# Autodesk Inventor assembly: 000-hand-grab-v1
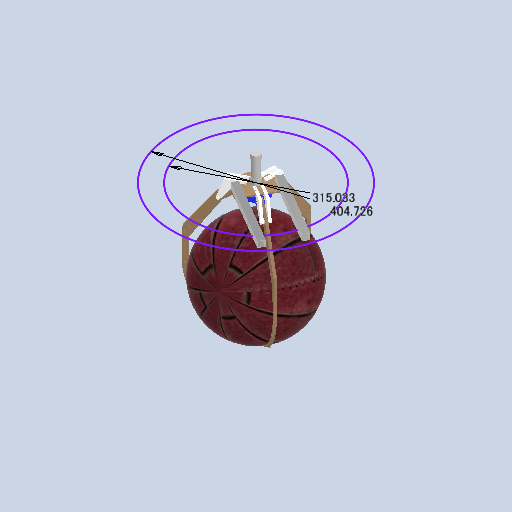
[picture p0: Inventor's stored thumbnail of the model, 512x512]
Saved by Autodesk Inventor 2025.1 (Build 291241000, 241)
## iProperties
Created: 2024-10-07
Part Number: 000-hand-grab-v1
Document SubType Name: Assembly
Designer: haruy
Author: haruy
## Documents named in this file (11)
- C:\Users\haruy\Documents\ロボコン\NHK2025\cad\nagahisa\hand\grab\000-hand-grab-v1.iam
- C:\Users\haruy\Documents\ロボコン\NHK2025\cad\nagahisa\hand\grab\hand-grab-v1-MDF-air-Base.ipt
- C:\Users\haruy\Documents\ロボコン\NHK2025\cad\nagahisa\hand\grab\hand-grab-v1-POM-link-F-1.ipt
- C:\Users\haruy\Documents\ロボコン\NHK2025\cad\nagahisa\hand\grab\hand-grab-v1-3DP-link-F-2.ipt
- C:\Users\haruy\Documents\ロボコン\NHK2025\cad\nagahisa\hand\grab\bearing-10-3.ipt
- C:\Users\haruy\Documents\ロボコン\NHK2025\cad\nagahisa\hand\grab\hand-grab-v1-POM-arm.ipt
- C:\Users\haruy\Documents\ロボコン\NHK2025\cad\nagahisa\hand\grab\C-SEFL683ZZ.ipt
- C:\Users\haruy\Documents\ロボコン\NHK2025\cad\nagahisa\hand\grab\E-NTBGT13-8.iam
- C:\Users\haruy\Documents\ロボコン\NHK2025\cad\basket-ball.ipt
- C:\Users\haruy\Documents\ロボコン\NHK2025\cad\000_parts\エアシリンダー\airclinder\CDJ2B16-15Z-B(0_1_0).iam
- C:\Users\haruy\Documents\ロボコン\NHK2025\cad\nagahisa\hand\grab\hand-grab-v1-ASP-arm-support.ipt
## Components (30 placed, 10 different names)
1. hand-grab-v1-MDF-air-Base:1 — 挿入:2, 挿入:3, 挿入:4, 挿入:5, 挿入:6, 挿入:7, 挿入:8, 挿入:9, 挿入:10, 挿入:11, 挿入:12, 挿入:13, 挿入:30, 挿入:32, 挿入:33, 挿入:34, 挿入:35
2. hand-grab-v1-POM-link-F-1:1 — 挿入:2, 挿入:3
3. hand-grab-v1-POM-link-F-1:2 — 挿入:4, 挿入:5
4. hand-grab-v1-POM-link-F-1:3 — 挿入:6, 挿入:7
5. hand-grab-v1-POM-link-F-1:4 — 挿入:8, 挿入:9
6. hand-grab-v1-POM-link-F-1:5 — 挿入:10, 挿入:11
7. hand-grab-v1-POM-link-F-1:6 — 挿入:12, 挿入:13, 角度:1, 挿入:29
8. hand-grab-v1-3DP-link-F-2:1 — 挿入:16, 挿入:18, 挿入:20, 角度:1, 挿入:31
9. bearing-10-3:1 — 挿入:15, 正接:3
10. bearing-10-3:2 — 挿入:15, 挿入:16
11. bearing-10-3:3
12. bearing-10-3:4 — 挿入:18
13. bearing-10-3:5 — 挿入:20
14. bearing-10-3:6
15. basket-ball:1 — 正接:4, 正接:5, 正接:6
16. CDJ2B16-15Z-B(0_1_0):1 [sub-assembly] — 挿入:30, 挿入:31
17. hand-grab-v1-ASP-arm-support:1 — 挿入:32, 挿入:34
18. hand-grab-v1-ASP-arm-support:2 — 挿入:33, 挿入:35
19. hand-grab-v1-POM-arm:1 — 挿入:26, 挿入:27, 挿入:28, 正接:3
20. E-NTBGT13-8:1 [sub-assembly] — 挿入:26, 正接:6
21. C-SEFL683ZZ:2 — 挿入:28
22. C-SEFL683ZZ:1 — 挿入:27, 挿入:29
23. hand-grab-v1-POM-arm:2
24. E-NTBGT13-8:2 [sub-assembly] — 正接:4
25. C-SEFL683ZZ:3
26. C-SEFL683ZZ:4
27. hand-grab-v1-POM-arm:3
28. E-NTBGT13-8:3 [sub-assembly] — 正接:5
29. C-SEFL683ZZ:5
30. C-SEFL683ZZ:6
## Component patterns: (3 elements, first: hand-grab-v1-POM-arm:1 + E-NTBGT13-8:1 + C-SEFL683ZZ:2 + C-SEFL683ZZ:1)
## Relationships (33: Insert 28, Tangent 4, Angle 1)
- 挿入:2 [Insert]: hand-grab-v1-MDF-air-Base:1 ↔ hand-grab-v1-POM-link-F-1:1
- 挿入:3 [Insert]: hand-grab-v1-MDF-air-Base:1 ↔ hand-grab-v1-POM-link-F-1:1
- 挿入:4 [Insert]: hand-grab-v1-MDF-air-Base:1 ↔ hand-grab-v1-POM-link-F-1:2
- 挿入:5 [Insert]: hand-grab-v1-MDF-air-Base:1 ↔ hand-grab-v1-POM-link-F-1:2
- 挿入:6 [Insert]: hand-grab-v1-MDF-air-Base:1 ↔ hand-grab-v1-POM-link-F-1:3
- 挿入:7 [Insert]: hand-grab-v1-MDF-air-Base:1 ↔ hand-grab-v1-POM-link-F-1:3
- 挿入:8 [Insert]: hand-grab-v1-MDF-air-Base:1 ↔ hand-grab-v1-POM-link-F-1:4
- 挿入:9 [Insert]: hand-grab-v1-MDF-air-Base:1 ↔ hand-grab-v1-POM-link-F-1:4
- 挿入:10 [Insert]: hand-grab-v1-MDF-air-Base:1 ↔ hand-grab-v1-POM-link-F-1:5
- 挿入:11 [Insert]: hand-grab-v1-MDF-air-Base:1 ↔ hand-grab-v1-POM-link-F-1:5
- 挿入:12 [Insert]: hand-grab-v1-MDF-air-Base:1 ↔ hand-grab-v1-POM-link-F-1:6
- 挿入:13 [Insert]: hand-grab-v1-MDF-air-Base:1 ↔ hand-grab-v1-POM-link-F-1:6
- 挿入:15 [Insert]: bearing-10-3:1 ↔ bearing-10-3:2
- 挿入:16 [Insert] (0.25 mm): hand-grab-v1-3DP-link-F-2:1 ↔ bearing-10-3:2
- [Insert]: bearing-10-3:3 ↔ bearing-10-3:4
- 挿入:18 [Insert] (0.25 mm): hand-grab-v1-3DP-link-F-2:1 ↔ bearing-10-3:4
- [Insert]: bearing-10-3:5 ↔ bearing-10-3:6
- 挿入:20 [Insert] (0.25 mm): hand-grab-v1-3DP-link-F-2:1 ↔ bearing-10-3:5
- 角度:1 [Angle] (0 deg): hand-grab-v1-POM-link-F-1:6 ↔ hand-grab-v1-3DP-link-F-2:1
- 挿入:26 [Insert]: hand-grab-v1-POM-arm:1 ↔ E-NTBGT13-8:1
- 挿入:27 [Insert]: hand-grab-v1-POM-arm:1 ↔ C-SEFL683ZZ:1
- 挿入:28 [Insert]: hand-grab-v1-POM-arm:1 ↔ C-SEFL683ZZ:2
- 挿入:29 [Insert] (0.2 mm): hand-grab-v1-POM-link-F-1:6 ↔ C-SEFL683ZZ:1
- 挿入:30 [Insert]: hand-grab-v1-MDF-air-Base:1 ↔ CDJ2B16-15Z-B(0_1_0):1
- 正接:3 [Tangent]: bearing-10-3:1 ↔ hand-grab-v1-POM-arm:1
- 正接:4 [Tangent]: basket-ball:1 ↔ E-NTBGT13-8:2
- 正接:5 [Tangent]: basket-ball:1 ↔ E-NTBGT13-8:3
- 正接:6 [Tangent]: basket-ball:1 ↔ E-NTBGT13-8:1
- 挿入:31 [Insert] (0.5 mm): hand-grab-v1-3DP-link-F-2:1 ↔ CDJ2B16-15Z-B(0_1_0):1
- 挿入:32 [Insert]: hand-grab-v1-MDF-air-Base:1 ↔ hand-grab-v1-ASP-arm-support:1
- 挿入:33 [Insert]: hand-grab-v1-MDF-air-Base:1 ↔ hand-grab-v1-ASP-arm-support:2
- 挿入:34 [Insert]: hand-grab-v1-MDF-air-Base:1 ↔ hand-grab-v1-ASP-arm-support:1
- 挿入:35 [Insert]: hand-grab-v1-MDF-air-Base:1 ↔ hand-grab-v1-ASP-arm-support:2
## Named parameters: d16_d14 = 0 mm, d18_d14 = 0 mm
